# Autodesk Inventor assembly: curved-+_plates
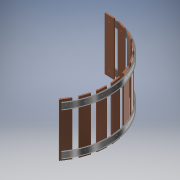
[picture p0: Inventor's stored thumbnail of the model, 180x180]
Saved by Autodesk Inventor 2019 (Build 230136000, 136)
## iProperties
Created: 2019-02-24
Part Number: curved-+_plates
Document SubType Name: Assembly
Designer: gaincarlo
Author: gaincarlo
## Documents named in this file (3)
- D:\Giancarlo Bacchio\Documenti\00 - Progetti\30-Inventor\LaPanca\curved-+_plates.iam
- D:\Giancarlo Bacchio\Documenti\00 - Progetti\30-Inventor\LaPanca\support2.ipt
- D:\Giancarlo Bacchio\Documenti\00 - Progetti\30-Inventor\LaPanca\doga_short.ipt
## Components (12 placed, 2 different names)
1. support2:1 — Mate:1, Mate:3
2. support2:2 — Mate:2
3. doga_short:1 — Mate:1, Mate:2, Mate:3
4. doga_short:2
5. doga_short:3
6. doga_short:4
7. doga_short:5
8. doga_short:6
9. doga_short:7
10. doga_short:8
11. doga_short:9
12. doga_short:10
## Component patterns: (2 elements, first: support2:1), (10 elements, first: doga_short:1)
## Relationships (3: Mate 3)
- Mate:1: support2:1 ↔ doga_short:1
- Mate:2: support2:2 ↔ doga_short:1
- Mate:3: support2:1 ↔ doga_short:1
